# Autodesk Inventor assembly: base_axis_8mm_2020-asm
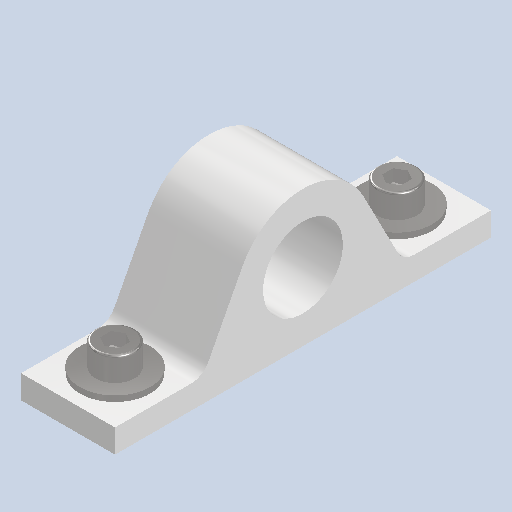
[picture p0: Inventor's stored thumbnail of the model, 512x512]
Saved by Autodesk Inventor 2024 (Build 280153000, 153)
## iProperties
Created: 2025-12-25
Part Number: base_axis_8mm_2020-asm
Document SubType Name: Assembly
Designer: schar
Author: schar
## Documents named in this file (5)
- C:\Users\schar\Desktop\projectBlueprint\AMSTS\hardware\base_axis_8mm_2020-asm.iam
- C:\Users\schar\Desktop\projectBlueprint\AMSTS\hardware\base_axis_8mm_2020.ipt
- C:\Users\schar\Documents\Inventor\Content Center Files\R2024\en-US\DIN 9021\DIN 9021 - 5,3.ipt
- C:\Users\schar\Documents\Inventor\Content Center Files\R2024\en-US\ISO 4762(1)\DIN EN ISO 4762 - M5 x 12.ipt
- C:\Users\schar\Desktop\projectBlueprint\AMSTS\hardware\tnut_m5_2020.ipt
## Components (7 placed, 4 different names)
1. base_axis_8mm_2020:1 — Mate:1, Mate:2, Mate:3, Mate:4, Mate:7, Mate:8, Rigid:1, Rigid:2
2. DIN 9021 5,3:1 — Mate:2, Mate:3, Mate:5
3. DIN 9021 5,3:2 — Mate:1, Mate:4, Mate:6
4. DIN EN ISO 4762 M5 x 12:1 — Mate:5, Mate:8
5. DIN EN ISO 4762 M5 x 12:2 — Mate:6, Mate:7
6. tnut_m5_2020:1 — Rigid:2
7. tnut_m5_2020:2 — Rigid:1
## Relationships (10: Mate 8, WeldJoint 2)
- Mate:1: base_axis_8mm_2020:1 ↔ DIN 9021 5,3:2
- Mate:2: base_axis_8mm_2020:1 ↔ DIN 9021 5,3:1
- Mate:3: base_axis_8mm_2020:1 ↔ DIN 9021 5,3:1
- Mate:4: base_axis_8mm_2020:1 ↔ DIN 9021 5,3:2
- Mate:5: DIN 9021 5,3:1 ↔ DIN EN ISO 4762 M5 x 12:1
- Mate:6: DIN 9021 5,3:2 ↔ DIN EN ISO 4762 M5 x 12:2
- Mate:7: base_axis_8mm_2020:1 ↔ DIN EN ISO 4762 M5 x 12:2
- Mate:8: base_axis_8mm_2020:1 ↔ DIN EN ISO 4762 M5 x 12:1
- Rigid:1 [WeldJoint] (-0.159 mm): base_axis_8mm_2020:1 ↔ tnut_m5_2020:2
- Rigid:2 [WeldJoint] (-0.159 mm): base_axis_8mm_2020:1 ↔ tnut_m5_2020:1
